# Autodesk Inventor assembly: pierna_ECO_v1.0
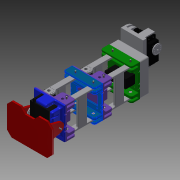
[picture p0: Inventor's stored thumbnail of the model, 180x180]
Saved by Autodesk Inventor 2015 (Build 190159000, 159)
## iProperties
Created: 2015-06-27
Part Number: pierna_ECO_v1.0
Document SubType Name: Assembly
Designer: Roberto
Author: Roberto
## Documents named in this file (13)
- D:\Piezas 3D\Pierna ECO\pierna_ECO_v1.0.iam
- D:\Piezas 3D\Pierna ECO\savox.ipt
- D:\Piezas 3D\Pierna ECO\horn.ipt
- D:\Piezas 3D\Pierna ECO\rodilla_superior.ipt
- C:\Users\Roberto\Documents\Inventor\Content Center Files\R2015\es-ES\GB 29.1-88\Bolt GB 29.1 M3 x 16.ipt
- D:\Piezas 3D\Pierna ECO\femur_actuado.ipt
- D:\Piezas 3D\Pierna ECO\femur_no_actuado.ipt
- D:\Piezas 3D\Pierna ECO\transversal.ipt
- D:\Piezas 3D\Pierna ECO\tobillo.ipt
- D:\Piezas 3D\Pierna ECO\pie.ipt
- D:\Piezas 3D\Pierna ECO\grapa.ipt
- D:\Piezas 3D\Pierna ECO\cadera_vertical.ipt
- D:\Piezas 3D\Pierna ECO\cadera_roll.ipt
## Components (40 placed, 12 different names)
1. pie:1 — Nivelación:11, Nivelación:15, Rígido:1, Ángulo:1
2. grapa:1 — Corredera:2
3. grapa:2 — Corredera:1
4. savox:4 — Nivelación:18, Coincidencia:20, Nivelación:19, De rotación:12
5. cadera_vertical:1 — Nivelación:20, Nivelación:22, Nivelación:23, Nivelación:24, Ángulo:2
6. horn:4 — De rotación:12, Rígido:2
7. cadera_roll:1 — Nivelación:22, Nivelación:23, Nivelación:24, Rígido:2, Ángulo:2, Coincidencia:21, Nivelación:25, Nivelación:26, Insertar:16
8. savox:5 — Coincidencia:21, Nivelación:25, Nivelación:26, De rotación:13
9. horn:5 — De rotación:13
10. Bolt GB/T 29.1-1988 M3x16:16 — Insertar:16
11. savox:2
12. horn:2
13. rodilla_superior:2 — Coincidencia:7, Nivelación:7, Nivelación:8
14. Bolt GB/T 29.1-1988 M3x16:8
15. Bolt GB/T 29.1-1988 M3x16:9
16. Bolt GB/T 29.1-1988 M3x16:10
17. femur_actuado:2 — Corredera:1
18. femur_no_actuado:2
19. transversal:2 — Nivelación:18, Coincidencia:20, Nivelación:19, Nivelación:20
20. Bolt GB/T 29.1-1988 M3x16:11
21. Bolt GB/T 29.1-1988 M3x16:12
22. Bolt GB/T 29.1-1988 M3x16:13
23. Bolt GB/T 29.1-1988 M3x16:14
24. savox:1 — De rotación:1, Coincidencia:1, Coincidencia:2, Coincidencia:3
25. horn:1 — De rotación:1, Nivelación:1, De rotación:2
26. rodilla_superior:1 — Coincidencia:1, Coincidencia:2, Insertar:1, Insertar:2, Insertar:3, Coincidencia:3, Nivelación:2, De rotación:4, Nivelación:3, Nivelación:9, Nivelación:16, Nivelación:17
27. Bolt GB/T 29.1-1988 M3x16:1 — Insertar:1
28. Bolt GB/T 29.1-1988 M3x16:2 — Insertar:2
29. Bolt GB/T 29.1-1988 M3x16:3 — Insertar:3
30. femur_actuado:1 — Nivelación:1, De rotación:2, De rotación:3, Corredera:2
31. femur_no_actuado:1 — Nivelación:2, De rotación:4, De rotación:5
32. transversal:1 — De rotación:3, De rotación:5, Insertar:4, Insertar:5, Insertar:6, Insertar:7, Nivelación:3, Coincidencia:7, Nivelación:7, Nivelación:8
33. Bolt GB/T 29.1-1988 M3x16:4 — Insertar:4
34. Bolt GB/T 29.1-1988 M3x16:5 — Insertar:5
35. Bolt GB/T 29.1-1988 M3x16:6 — Insertar:6
36. Bolt GB/T 29.1-1988 M3x16:7 — Insertar:7
37. tobillo:1 — Nivelación:9, Coincidencia:8, Coincidencia:9, Nivelación:10, Insertar:15, Nivelación:15, Nivelación:16, Nivelación:17, Ángulo:1
38. savox:3 — Coincidencia:8, Coincidencia:9, Nivelación:10, De rotación:11
39. horn:3 — De rotación:11, Nivelación:11, Rígido:1
40. Bolt GB/T 29.1-1988 M3x16:15 — Insertar:15
## Relationships (68: Flush 22, Insert 16, RevoluteJoint 13, Mate 11, WeldJoint 2, Angle 2, TranslationJoint 2)
- De rotación:1 [RevoluteJoint]: savox:1 ↔ horn:1
- Coincidencia:1 [Mate] (1 mm): savox:1 ↔ rodilla_superior:1
- Coincidencia:2 [Mate] (0.5 mm): savox:1 ↔ rodilla_superior:1
- Insertar:1: rodilla_superior:1 ↔ Bolt GB/T 29.1-1988 M3x16:1
- Insertar:2: rodilla_superior:1 ↔ Bolt GB/T 29.1-1988 M3x16:2
- Insertar:3: rodilla_superior:1 ↔ Bolt GB/T 29.1-1988 M3x16:3
- Nivelación:1 [Flush]: horn:1 ↔ femur_actuado:1
- Coincidencia:3 [Mate] (0.5 mm): savox:1 ↔ rodilla_superior:1
- Nivelación:2 [Flush] (0.25 mm): rodilla_superior:1 ↔ femur_no_actuado:1
- De rotación:2 [RevoluteJoint]: horn:1 ↔ femur_actuado:1
- De rotación:3 [RevoluteJoint] (0.25 mm): femur_actuado:1 ↔ transversal:1
- De rotación:4 [RevoluteJoint] (-0.25 mm): rodilla_superior:1 ↔ femur_no_actuado:1
- De rotación:5 [RevoluteJoint] (-0.35 mm): femur_no_actuado:1 ↔ transversal:1
- Insertar:4: transversal:1 ↔ Bolt GB/T 29.1-1988 M3x16:4
- Insertar:5: transversal:1 ↔ Bolt GB/T 29.1-1988 M3x16:5
- Insertar:6: transversal:1 ↔ Bolt GB/T 29.1-1988 M3x16:6
- Insertar:7: transversal:1 ↔ Bolt GB/T 29.1-1988 M3x16:7
- Nivelación:3 [Flush]: rodilla_superior:1 ↔ transversal:1
- [RevoluteJoint]: savox:2 ↔ horn:2
- [Mate] (1 mm): savox:2 ↔ rodilla_superior:2
- [Mate] (0.5 mm): savox:2 ↔ rodilla_superior:2
- [Insert]: rodilla_superior:2 ↔ Bolt GB/T 29.1-1988 M3x16:8
- [Insert]: rodilla_superior:2 ↔ Bolt GB/T 29.1-1988 M3x16:9
- [Insert]: rodilla_superior:2 ↔ Bolt GB/T 29.1-1988 M3x16:10
- [Flush]: horn:2 ↔ femur_actuado:2
- [Mate] (0.5 mm): savox:2 ↔ rodilla_superior:2
- [Flush] (0.25 mm): rodilla_superior:2 ↔ femur_no_actuado:2
- [RevoluteJoint]: horn:2 ↔ femur_actuado:2
- [RevoluteJoint] (0.25 mm): femur_actuado:2 ↔ transversal:2
- [RevoluteJoint] (-0.25 mm): rodilla_superior:2 ↔ femur_no_actuado:2
- [RevoluteJoint] (-0.35 mm): femur_no_actuado:2 ↔ transversal:2
- [Insert]: transversal:2 ↔ Bolt GB/T 29.1-1988 M3x16:11
- [Insert]: transversal:2 ↔ Bolt GB/T 29.1-1988 M3x16:12
- [Insert]: transversal:2 ↔ Bolt GB/T 29.1-1988 M3x16:13
- [Insert]: transversal:2 ↔ Bolt GB/T 29.1-1988 M3x16:14
- [Flush]: rodilla_superior:2 ↔ transversal:2
- Coincidencia:7 [Mate]: rodilla_superior:2 ↔ transversal:1
- Nivelación:7 [Flush]: rodilla_superior:2 ↔ transversal:1
- Nivelación:8 [Flush]: rodilla_superior:2 ↔ transversal:1
- Nivelación:9 [Flush]: rodilla_superior:1 ↔ tobillo:1
- Coincidencia:8 [Mate] (0.5 mm): tobillo:1 ↔ savox:3
- Coincidencia:9 [Mate] (-49 mm): tobillo:1 ↔ savox:3
- Nivelación:10 [Flush] (15 mm): tobillo:1 ↔ savox:3
- De rotación:11 [RevoluteJoint]: savox:3 ↔ horn:3
- Insertar:15: tobillo:1 ↔ Bolt GB/T 29.1-1988 M3x16:15
- Nivelación:11 [Flush]: pie:1 ↔ horn:3
- Nivelación:15 [Flush] (0.5 mm): pie:1 ↔ tobillo:1
- Rígido:1 [WeldJoint]: pie:1 ↔ horn:3
- Nivelación:16 [Flush]: rodilla_superior:1 ↔ tobillo:1
- Nivelación:17 [Flush]: rodilla_superior:1 ↔ tobillo:1
- Ángulo:1 [Angle] (360 deg): pie:1 ↔ tobillo:1
- Corredera:1 [TranslationJoint]: grapa:2 ↔ femur_actuado:2
- Corredera:2 [TranslationJoint]: grapa:1 ↔ femur_actuado:1
- Nivelación:18 [Flush] (-20 mm): savox:4 ↔ transversal:2
- Coincidencia:20 [Mate] (-46.5 mm): savox:4 ↔ transversal:2
- Nivelación:19 [Flush] (2 mm): savox:4 ↔ transversal:2
- Nivelación:20 [Flush]: cadera_vertical:1 ↔ transversal:2
- De rotación:12 [RevoluteJoint] (0.5 mm): savox:4 ↔ horn:4
- Nivelación:22 [Flush] (0.5 mm): cadera_vertical:1 ↔ cadera_roll:1
- Nivelación:23 [Flush]: cadera_vertical:1 ↔ cadera_roll:1
- Nivelación:24 [Flush] (0.5 mm): cadera_vertical:1 ↔ cadera_roll:1
- Rígido:2 [WeldJoint] (-0.3 mm): horn:4 ↔ cadera_roll:1
- Ángulo:2 [Angle] (0 deg): cadera_vertical:1 ↔ cadera_roll:1
- Coincidencia:21 [Mate] (0.5 mm): cadera_roll:1 ↔ savox:5
- Nivelación:25 [Flush]: cadera_roll:1 ↔ savox:5
- Nivelación:26 [Flush] (-2 mm): cadera_roll:1 ↔ savox:5
- De rotación:13 [RevoluteJoint] (0.5 mm): savox:5 ↔ horn:5
- Insertar:16: cadera_roll:1 ↔ Bolt GB/T 29.1-1988 M3x16:16
## Named parameters: d25_d17 = 90 deg, d26_d18 = 0 mm, d27_d19 = 0 mm, d28_d20 = 0 mm, d29_d21 = 0 mm, d30_d24 = 0 mm, d31_d9 = 0.25 mm, d32_d10 = 0 mm, d33_d11 = 71.903461 deg, d34_d12 = 0.25 mm, d35_d13 = 180 deg, d36_d14 = -0.25 mm, d37_d15 = 0 deg, d38_d16 = -0.35 mm, d39_d7 = 0 mm, d40_d8 = 0.5 mm, d41_d0 = 0 mm, d42_d1 = 161.903461 deg, d43_d2 = 1 mm, d44_d3 = 0.5 mm, d45_d4 = 0 mm, d46_d5 = 0 mm, d47_d6 = 0 mm
